# Autodesk Inventor assembly: ass_sucrose
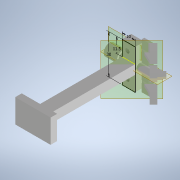
[picture p0: Inventor's stored thumbnail of the model, 180x180]
Saved by Autodesk Inventor 2020.1 (Build 241239000, 239)
## iProperties
Created: 2019-07-31
Part Number: ass_sucrose
Document SubType Name: Assembly
Designer: Chang Ko
Author: Chang Ko
## Documents named in this file (3)
- C:\Users\Chang Ko\Documents\연구\inventor project\ass_sucrose.iam
- C:\Users\Chang Ko\Documents\연구\inventor project\LickSensorMount.ipt
- C:\Users\Chang Ko\Documents\연구\inventor project\sucrose training holder.ipt
## Components (2 placed, 2 different names)
1. LickSensorMount:1 — 강체:1
2. sucrose training holder:1 — 강체:1
## Relationships (1: WeldJoint 1)
- 강체:1 [WeldJoint]: LickSensorMount:1 ↔ sucrose training holder:1
